# Autodesk Inventor assembly: casting pattern
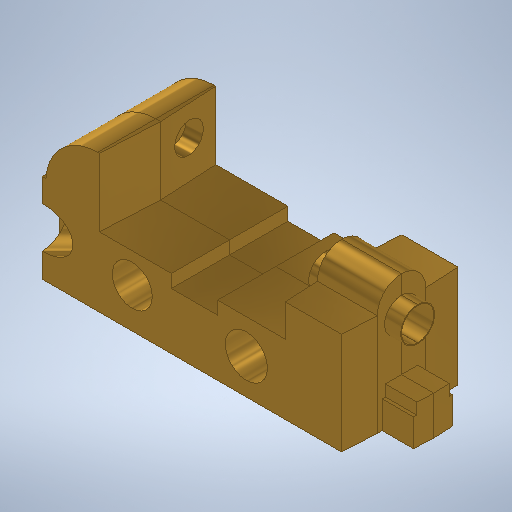
[picture p0: Inventor's stored thumbnail of the model, 512x512]
Saved by Autodesk Inventor 2025.2 (Build 292293000, 293)
## iProperties
Created: 2024-05-01
Part Number: casting pattern
Document SubType Name: Assembly
Designer: abdal
Author: abdal
## Documents named in this file (3)
- C:\Users\abdal\Desktop\FINAL MECHANICAL MOVMENT WITH STAND\casting pattern\casting pattern\casting pattern.iam
- C:\Users\abdal\Desktop\FINAL MECHANICAL MOVMENT WITH STAND\casting pattern\casting pattern\Casting Project right.ipt
- C:\Users\abdal\Desktop\FINAL MECHANICAL MOVMENT WITH STAND\casting pattern\casting pattern\Casting Project left.ipt
## Components (2 placed, 2 different names)
1. Casting Project right:1
2. Casting Project left:1 — Mate:1, Angle:1, Mate:2, Angle:2
## Relationships (4: Mate 2, Angle 2)
- Mate:1: Casting Project left:1
- Angle:1 (0 deg): Casting Project left:1
- Mate:2: Casting Project left:1
- Angle:2 (-45 deg): Casting Project left:1
